# Autodesk Inventor assembly: TestMergerWseat
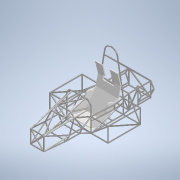
[picture p0: Inventor's stored thumbnail of the model, 180x180]
Saved by Autodesk Inventor 2021 (Build 250183000, 183)
## iProperties
Created: 2020-10-11
Part Number: TestMergerWseat
Document SubType Name: Assembly
Designer: qv17m
_SolveAssemblyDoc: Frame Generator Solve Assembly
_Version: 25.0.0
Author: qv17m
## Documents named in this file (8)
- C:\Users\atwaterh\Documents\Inventor\FromBert\TestMerger - Copy\TestMergerWseat.iam
- C:\Users\atwaterh\Documents\Inventor\FromBert\TestMerger - Copy\FSAE_Frame.0007.ipt
- C:\Users\atwaterh\Documents\Inventor\FromBert\TestMerger - Copy\DesignReviewOct_10 - Copy.ipt
- C:\Users\atwaterh\Documents\Inventor\FromBert\TestMerger - Copy\Frame\Frame.iam
- C:\Users\atwaterh\Documents\Inventor\FromBert\TestMerger - Copy\Frame\Seat3DSketch.ipt
- C:\Users\atwaterh\Documents\Inventor\FromBert\TestMerger - Copy\Frame\Seat tab to frame mount.ipt
- C:\Users\atwaterh\Documents\Inventor\FromBert\TestMerger - Copy\Frame\Seat tabsnew.ipt
- C:\Users\atwaterh\Documents\Inventor\FromBert\TestMerger - Copy\Frame\harness attachments.ipt
## Components (13 placed, 7 different names)
1. FSAE_Frame.0007:1 — Mate:1
2. DesignReviewOct_10 - Copy:1 — Mate:1
3. Frame:1 [sub-assembly] — Mate:26, Mate:34, Mate:44, Mate:45, Mate:46, Mate:47, Mate:48, Mate:49, Mate:50, Mate:51, Mate:57, Mate:58, Mate:59, Mate:60, Angle:1, Angle:2, Mate:61, Mate:62, Angle:3
4. Seat3DSketch:2 — Mate:53, Mate:54, Mate:55
5. Seat tab to frame mount:1 — Mate:41, Mate:42, Mate:44, Mate:47, Mate:50, Mate:51
6. Seat tab to frame mount:2 — Mate:40, Mate:48, Mate:49
7. Seat tab to frame mount:3 — Mate:45, Mate:46, Mate:52, Mate:56
8. Seat tab to frame mount:4 — Mate:26, Mate:34, Mate:38, Mate:39
9. Seat tabsnew:1 — Mate:38, Mate:39, Mate:40, Mate:53, Mate:54, Mate:55
10. Seat tabsnew:2 — Mate:41, Mate:42, Mate:52, Mate:56
11. harness attachments:1 — Mate:57, Mate:58, Angle:2
12. harness attachments:2 — Mate:59, Mate:60, Angle:1
13. harness attachments:3 — Mate:61, Mate:62, Angle:3
## Relationships (30: Mate 27, Angle 3)
- Mate:1: FSAE_Frame.0007:1 ↔ DesignReviewOct_10 - Copy:1
- Mate:26: Frame:1 ↔ Seat tab to frame mount:4
- Mate:34: Frame:1 ↔ Seat tab to frame mount:4
- Mate:38 (6.35 mm): Seat tab to frame mount:4 ↔ Seat tabsnew:1
- Mate:39: Seat tab to frame mount:4 ↔ Seat tabsnew:1
- Mate:40: Seat tab to frame mount:2 ↔ Seat tabsnew:1
- Mate:41: Seat tab to frame mount:1 ↔ Seat tabsnew:2
- Mate:42: Seat tab to frame mount:1 ↔ Seat tabsnew:2
- Mate:44: Frame:1 ↔ Seat tab to frame mount:1
- Mate:45: Frame:1 ↔ Seat tab to frame mount:3
- Mate:46: Frame:1 ↔ Seat tab to frame mount:3
- Mate:47: Frame:1 ↔ Seat tab to frame mount:1
- Mate:48: Frame:1 ↔ Seat tab to frame mount:2
- Mate:49: Frame:1 ↔ Seat tab to frame mount:2
- Mate:50: Frame:1 ↔ Seat tab to frame mount:1
- Mate:51: Frame:1 ↔ Seat tab to frame mount:1
- Mate:52 (6.35 mm): Seat tab to frame mount:3 ↔ Seat tabsnew:2
- Mate:53: Seat3DSketch:2 ↔ Seat tabsnew:1
- Mate:54: Seat3DSketch:2 ↔ Seat tabsnew:1
- Mate:55 (-6.35 mm): Seat3DSketch:2 ↔ Seat tabsnew:1
- Mate:56: Seat tab to frame mount:3 ↔ Seat tabsnew:2
- Mate:57: Frame:1 ↔ harness attachments:1
- Mate:58: Frame:1 ↔ harness attachments:1
- Mate:59: Frame:1 ↔ harness attachments:2
- Mate:60: Frame:1 ↔ harness attachments:2
- Angle:1 (90 deg): Frame:1 ↔ harness attachments:2
- Angle:2 (90 deg): Frame:1 ↔ harness attachments:1
- Mate:61: Frame:1 ↔ harness attachments:3
- Mate:62: Frame:1 ↔ harness attachments:3
- Angle:3 (90 deg): Frame:1 ↔ harness attachments:3
